# Autodesk Inventor assembly: Bed Mount
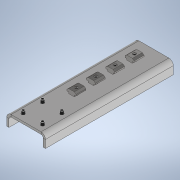
[picture p0: Inventor's stored thumbnail of the model, 180x180]
Saved by Autodesk Inventor 2022 (Build 260153000, 153)
## iProperties
Created: 2022-03-12
Part Number: Bed Mount
Document SubType Name: Assembly
Designer: Nick
Author: Nick
## Documents named in this file (6)
- Y:\Projects\Bibble0\SubAsm\Bed Mount.iam
- Y:\Projects\Bibble0\Hardware\M3 x 6 mm SHCS.ipt
- Y:\Projects\Bibble0\Sheet Metal\Bed Mount.ipt
- Y:\Projects\Bibble0\Hardware\M3 Washer.ipt
- Y:\Projects\Bibble0\Hardware\M3 T-Slot Nut.ipt
- Y:\Projects\Bibble0\Hardware\M3 x 8 mm SHCS.ipt
## Components (21 placed, 5 different names)
1. M3 x 6 mm SHCS:1 — Insert:1
2. Bed Mount:2 — Insert:9, Insert:10, Insert:11, Insert:12, Insert:17, Insert:18, Insert:19, Insert:20, Insert:21, Insert:22, Insert:23, Insert:24, Angle:4
3. M3 Washer:1 — Insert:1, Insert:9
4. M3 x 6 mm SHCS:2
5. M3 Washer:2 — Insert:10
6. M3 x 6 mm SHCS:3
7. M3 Washer:3 — Insert:12
8. M3 x 6 mm SHCS:4
9. M3 Washer:4 — Insert:11
10. M3 T-Slot Nut:1 — Insert:21, Angle:1
11. M3 T-Slot Nut:2 — Insert:22, Angle:1, Angle:2
12. M3 T-Slot Nut:3 — Insert:23, Angle:2, Angle:3
13. M3 T-Slot Nut:4 — Insert:24, Angle:3, Angle:4
14. M3 x 8 mm SHCS:1 — Insert:13
15. M3 Washer:5 — Insert:13, Insert:17
16. M3 x 8 mm SHCS:2
17. M3 Washer:6 — Insert:18
18. M3 x 8 mm SHCS:3
19. M3 Washer:7 — Insert:19
20. M3 x 8 mm SHCS:4
21. M3 Washer:8 — Insert:20
## Relationships (24: Insert 20, Angle 4)
- Insert:1: M3 x 6 mm SHCS:1 ↔ M3 Washer:1
- [Insert]: M3 x 6 mm SHCS:2 ↔ M3 Washer:2
- [Insert]: M3 x 6 mm SHCS:3 ↔ M3 Washer:3
- [Insert]: M3 x 6 mm SHCS:4 ↔ M3 Washer:4
- Insert:9: Bed Mount:2 ↔ M3 Washer:1
- Insert:10: Bed Mount:2 ↔ M3 Washer:2
- Insert:11: Bed Mount:2 ↔ M3 Washer:4
- Insert:12: Bed Mount:2 ↔ M3 Washer:3
- Insert:13: M3 x 8 mm SHCS:1 ↔ M3 Washer:5
- [Insert]: M3 x 8 mm SHCS:2 ↔ M3 Washer:6
- [Insert]: M3 x 8 mm SHCS:3 ↔ M3 Washer:7
- [Insert]: M3 x 8 mm SHCS:4 ↔ M3 Washer:8
- Insert:17: Bed Mount:2 ↔ M3 Washer:5
- Insert:18: Bed Mount:2 ↔ M3 Washer:6
- Insert:19: Bed Mount:2 ↔ M3 Washer:7
- Insert:20: Bed Mount:2 ↔ M3 Washer:8
- Insert:21 (1.5 mm): Bed Mount:2 ↔ M3 T-Slot Nut:1
- Insert:22 (1.5 mm): Bed Mount:2 ↔ M3 T-Slot Nut:2
- Insert:23 (1.5 mm): Bed Mount:2 ↔ M3 T-Slot Nut:3
- Insert:24 (1.5 mm): Bed Mount:2 ↔ M3 T-Slot Nut:4
- Angle:1 (0 deg): M3 T-Slot Nut:1 ↔ M3 T-Slot Nut:2
- Angle:2 (0 deg): M3 T-Slot Nut:2 ↔ M3 T-Slot Nut:3
- Angle:3 (0 deg): M3 T-Slot Nut:3 ↔ M3 T-Slot Nut:4
- Angle:4 (0 deg): Bed Mount:2 ↔ M3 T-Slot Nut:4
## Named parameters: d1_d0 = 0 mm, d2_d0 = 0 mm, d3_d0 = 0 mm, d17_d16 = 0 mm, d18_d16 = 0 mm, d19_d16 = 0 mm
